# Autodesk Inventor assembly: rail_carrier
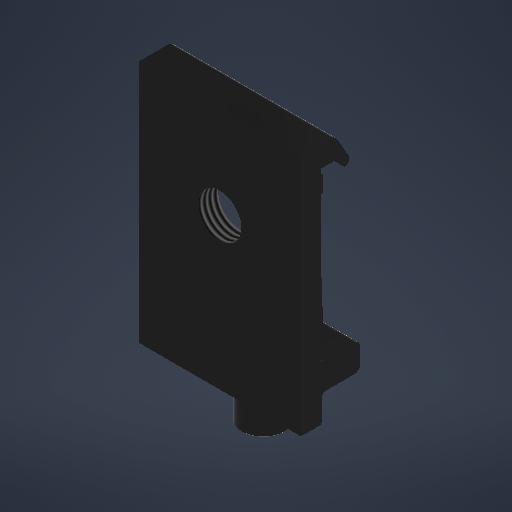
[picture p0: Inventor's stored thumbnail of the model, 512x512]
Saved by Autodesk Inventor 2026 (Build 300175050, 175E)
## iProperties
Created: 2025-07-09
Part Number: rail_carrier
Document SubType Name: Assembly
Designer: jin20
Author: jin20
## Documents named in this file (4)
- C:\Users\jin20\Documents\装置CAD\RamanSystem\Stage\rail_carrier\rail_carrier.iam
- C:\Users\jin20\Documents\装置CAD\RamanSystem\Stage\rail_carrier\carrier_base.ipt
- C:\Users\jin20\Documents\装置CAD\RamanSystem\Stage\rail_carrier\carrier_holder.ipt
- C:\Users\jin20\Documents\装置CAD\RamanSystem\Stage\rail_carrier\carrier_handle.ipt
## Components (3 placed, 3 different names)
1. carrier_base:1 — 挿入:1
2. carrier_holder:1 — 挿入:1, 挿入:2
3. carrier_handle:1 — 挿入:2
## Relationships (2: Insert 2)
- 挿入:1 [Insert] (1.9 mm): carrier_base:1 ↔ carrier_holder:1
- 挿入:2 [Insert]: carrier_holder:1 ↔ carrier_handle:1
